# Autodesk Inventor assembly: HalfChassisAssem_MIR
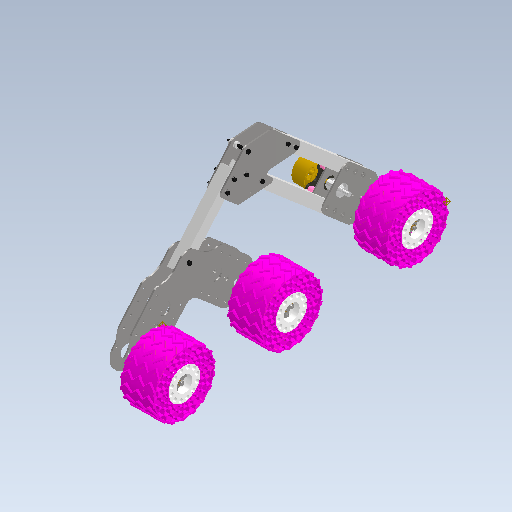
[picture p0: Inventor's stored thumbnail of the model, 512x512]
Saved by Autodesk Inventor 2023 (Build 270158000, 158)
## iProperties
Created: 2023-04-06
Part Number: HalfChassisAssem_MIR
Document SubType Name: Assembly
Designer: Dave
Mass: 5362.71 g
Surface Area: 20188.6 cm^2
Volume: 2426.63 cm^3
Density: 2.20995 g/cm^3
Author: Dave
## Documents named in this file (13)
- C:\Users\Dave\Documents\GitHub\BehrendURCMechanical\CAD\Chassis V3\HalfChassisAssem_MIR.iam
- C:\Users\Dave\Documents\GitHub\BehrendURCMechanical\CAD\Chassis V3\L3 Gearbox Assembly_MIR.iam
- C:\Users\Dave\Documents\GitHub\BehrendURCMechanical\CAD\Chassis V3\L1 Gearbox Assembly_MIR.iam
- C:\Users\Dave\Documents\GitHub\BehrendURCMechanical\CAD\Chassis V3\HipPivotPlate_MIR.ipt
- C:\Users\Dave\Documents\GitHub\BehrendURCMechanical\CAD\Chassis V3\aluminumextrusiontool\aluminumextrusiontool-17-10.6in.ipt
- C:\Users\Dave\Documents\GitHub\BehrendURCMechanical\CAD\Chassis V3\aluminumextrusiontool.ipt
- C:\Users\Dave\Documents\GitHub\BehrendURCMechanical\CAD\Chassis V3\aluminumextrusiontool\aluminumextrusiontool-17-7.9.ipt
- C:\Users\Dave\Documents\GitHub\BehrendURCMechanical\CAD\Chassis V3\Wheel\WheelAssembly_v8_MIR.iam
- C:\Users\Dave\Documents\GitHub\BehrendURCMechanical\CAD\Chassis V3\aluminumextrusiontool\aluminumextrusiontool-17-13.31255in.ipt
- C:\Users\Dave\Documents\GitHub\BehrendURCMechanical\CAD\Chassis V3\Pivot Files and Assembly\PivotAssembly_MIR.iam
- C:\Users\Dave\Documents\GitHub\BehrendURCMechanical\CAD\Chassis V3\91333A140_Low-Strength Steel Nylon-Insert Locknut_MIR.ipt
- C:\Users\Dave\Documents\GitHub\BehrendURCMechanical\CAD\Chassis V3\90107A011_316 Stainless Steel Washer_MIR.ipt
- C:\Users\Dave\Documents\GitHub\BehrendURCMechanical\CAD\Chassis V3\Bolt Nut Washer assem_MIR.iam
## Components (20 placed, 11 different names)
1. L3 Gearbox Assembly_MIR:1 [sub-assembly] — Mate:4, Mate:10, Tangent:2, Insert:1
2. L1 Gearbox Assembly_MIR:1 [sub-assembly] — Flush:3, Flush:6, Mate:1, Flush:2, Mate:3, Flush:7, Mate:2, Flush:10, Mate:7, Flush:13, Mate:11
3. HipPivotPlate_MIR:1 — Flush:3, Flush:5, Flush:4, Mate:5, Insert:4
4. HipPivotPlate_MIR:2 — Flush:9, Mate:6, Mate:4, Flush:6, Mate:1, Flush:5, Flush:4, Flush:2, Tangent:1, Flush:8, Insert:6, Insert:7, Insert:9, Insert:10, Insert:11, Insert:12, Insert:14
5. aluminumextrusiontool-17-10.6in:1 — Mate:3, Flush:7, Mate:2
6. aluminumextrusiontool-17-7.9:2 — Mate:10, Tangent:2, Tangent:1, Flush:8, Mate:5
7. WheelAssembly_v8_MIR:1 [sub-assembly] — Flush:10, Mate:7
8. WheelAssembly_v8_MIR:2 [sub-assembly] — Flush:14
9. WheelAssembly_v8_MIR:3 [sub-assembly] — Flush:14
10. aluminumextrusiontool-17-13.31255in:3 — Flush:13, Mate:11
11. PivotAssembly_MIR:1 [sub-assembly] — Insert:1
12. PivotAssembly_MIR:2 [sub-assembly] — Insert:6
13. 91333A140_Low-Strength Steel Nylon-Insert Locknut_MIR:1 — Insert:5
14. 90107A011_316 Stainless Steel Washer_MIR:1 — Insert:5, Insert:4
15. Bolt Nut Washer assem_MIR:1 [sub-assembly] — Insert:7
16. Bolt Nut Washer assem_MIR:2 [sub-assembly] — Insert:9
17. Bolt Nut Washer assem_MIR:3 [sub-assembly] — Insert:10
18. Bolt Nut Washer assem_MIR:4 [sub-assembly] — Insert:11
19. Bolt Nut Washer assem_MIR:5 [sub-assembly] — Insert:12
20. Bolt Nut Washer assem_MIR:6 [sub-assembly] — Insert:14
## Relationships (32: Flush 11, Insert 10, Mate 9, Tangent 2)
- Flush:3: L1 Gearbox Assembly_MIR:1 ↔ HipPivotPlate_MIR:1
- Flush:9: HipPivotPlate_MIR:2
- Mate:6: HipPivotPlate_MIR:2
- Mate:4 (216 mm): L3 Gearbox Assembly_MIR:1 ↔ HipPivotPlate_MIR:2
- Flush:6: L1 Gearbox Assembly_MIR:1 ↔ HipPivotPlate_MIR:2
- Mate:1 (396 mm): L1 Gearbox Assembly_MIR:1 ↔ HipPivotPlate_MIR:2
- Flush:5: HipPivotPlate_MIR:1 ↔ HipPivotPlate_MIR:2
- Flush:4: HipPivotPlate_MIR:1 ↔ HipPivotPlate_MIR:2
- Flush:2: L1 Gearbox Assembly_MIR:1 ↔ HipPivotPlate_MIR:2
- Mate:3 (-76.2 mm): L1 Gearbox Assembly_MIR:1 ↔ aluminumextrusiontool-17-10.6in:1
- Flush:7: L1 Gearbox Assembly_MIR:1 ↔ aluminumextrusiontool-17-10.6in:1
- Mate:2: L1 Gearbox Assembly_MIR:1 ↔ aluminumextrusiontool-17-10.6in:1
- Mate:10: L3 Gearbox Assembly_MIR:1 ↔ aluminumextrusiontool-17-7.9:2
- Tangent:2 (6.35 mm): L3 Gearbox Assembly_MIR:1 ↔ aluminumextrusiontool-17-7.9:2
- Tangent:1 (12.7 mm): HipPivotPlate_MIR:2 ↔ aluminumextrusiontool-17-7.9:2
- Flush:8: HipPivotPlate_MIR:2 ↔ aluminumextrusiontool-17-7.9:2
- Mate:5: HipPivotPlate_MIR:1 ↔ aluminumextrusiontool-17-7.9:2
- Flush:10: L1 Gearbox Assembly_MIR:1 ↔ WheelAssembly_v8_MIR:1
- Mate:7: L1 Gearbox Assembly_MIR:1 ↔ WheelAssembly_v8_MIR:1
- Flush:14: WheelAssembly_v8_MIR:2 ↔ WheelAssembly_v8_MIR:3
- Flush:13: L1 Gearbox Assembly_MIR:1 ↔ aluminumextrusiontool-17-13.31255in:3
- Mate:11: L1 Gearbox Assembly_MIR:1 ↔ aluminumextrusiontool-17-13.31255in:3
- Insert:1: L3 Gearbox Assembly_MIR:1 ↔ PivotAssembly_MIR:1
- Insert:6: HipPivotPlate_MIR:2 ↔ PivotAssembly_MIR:2
- Insert:5: 91333A140_Low-Strength Steel Nylon-Insert Locknut_MIR:1 ↔ 90107A011_316 Stainless Steel Washer_MIR:1
- Insert:4: HipPivotPlate_MIR:1 ↔ 90107A011_316 Stainless Steel Washer_MIR:1
- Insert:7: HipPivotPlate_MIR:2 ↔ Bolt Nut Washer assem_MIR:1
- Insert:9: HipPivotPlate_MIR:2 ↔ Bolt Nut Washer assem_MIR:2
- Insert:10: HipPivotPlate_MIR:2 ↔ Bolt Nut Washer assem_MIR:3
- Insert:11: HipPivotPlate_MIR:2 ↔ Bolt Nut Washer assem_MIR:4
- Insert:12: HipPivotPlate_MIR:2 ↔ Bolt Nut Washer assem_MIR:5
- Insert:14: HipPivotPlate_MIR:2 ↔ Bolt Nut Washer assem_MIR:6
